# Autodesk Inventor assembly: OBUDOWA TYLNA + PRZEDNIA + BLACHA ZE ZŁĄCZAMI
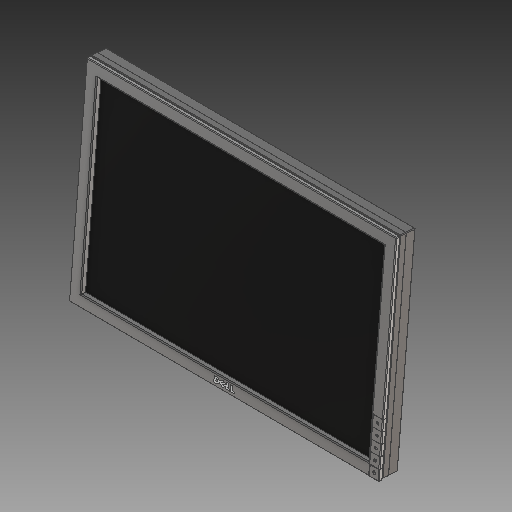
[picture p0: Inventor's stored thumbnail of the model, 512x512]
Saved by Autodesk Inventor 2017 SP1 (Build 210196100, 196)
## iProperties
Created: 2021-03-07
Part Number: OBUDOWA TYLNA + PRZEDNIA + BLACHA ZE ZŁĄCZAMI
Document SubType Name: Assembly
Designer: Administrator
Author: Administrator
## Documents named in this file (4)
- D:\PRYWATNE\PROJEKTY\POKÓJ\URZĄDZENIA PERYFERYJNE\DELL 1909Wf\OBUDOWA TYLNA + PRZEDNIA + BLACHA ZE ZŁĄCZAMI.iam
- D:\PRYWATNE\PROJEKTY\POKÓJ\URZĄDZENIA PERYFERYJNE\DELL 1909Wf\OBUDOWA TYLNA MONITORA + ZŁĄCZA.iam
- D:\PRYWATNE\PROJEKTY\POKÓJ\URZĄDZENIA PERYFERYJNE\DELL 1909Wf\BLACHA+ZŁĄCZA.iam
- D:\PRYWATNE\PROJEKTY\POKÓJ\URZĄDZENIA PERYFERYJNE\DELL 1909Wf\OBUDOWA PRZEDNIA + PRZYCISKI + MATRYCA.iam
## Components (3 placed, 3 different names)
1. OBUDOWA TYLNA MONITORA + ZŁĄCZA:1 [sub-assembly] — Zestawiający:1, Zestawiający:2, Zestawiający:3, Zestawiający:4, Równoległy:1, Równoległy:2
2. BLACHA+ZŁĄCZA:1 [sub-assembly] — Zestawiający:1, Zestawiający:2, Zestawiający:3
3. OBUDOWA PRZEDNIA + PRZYCISKI + MATRYCA:1 [sub-assembly] — Zestawiający:4, Równoległy:1, Równoległy:2
## Relationships (6: Mate 4, Flush 2)
- Zestawiający:1 [Mate] (2 mm): OBUDOWA TYLNA MONITORA + ZŁĄCZA:1 ↔ BLACHA+ZŁĄCZA:1
- Zestawiający:2 [Mate] (2 mm): OBUDOWA TYLNA MONITORA + ZŁĄCZA:1 ↔ BLACHA+ZŁĄCZA:1
- Zestawiający:3 [Mate]: OBUDOWA TYLNA MONITORA + ZŁĄCZA:1 ↔ BLACHA+ZŁĄCZA:1
- Zestawiający:4 [Mate]: OBUDOWA TYLNA MONITORA + ZŁĄCZA:1 ↔ OBUDOWA PRZEDNIA + PRZYCISKI + MATRYCA:1
- Równoległy:1 [Flush] (1.5 mm): OBUDOWA TYLNA MONITORA + ZŁĄCZA:1 ↔ OBUDOWA PRZEDNIA + PRZYCISKI + MATRYCA:1
- Równoległy:2 [Flush] (1.5 mm): OBUDOWA TYLNA MONITORA + ZŁĄCZA:1 ↔ OBUDOWA PRZEDNIA + PRZYCISKI + MATRYCA:1
